# Autodesk Inventor assembly: Seed hand
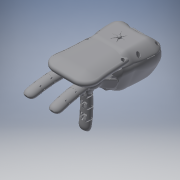
[picture p0: Inventor's stored thumbnail of the model, 180x180]
Saved by Autodesk Inventor 2016 (Build 200138000, 138)
## iProperties
Created: 2016-03-09
Part Number: Seed hand
Document SubType Name: Assembly
Designer: Ironic
Author: Ironic
## Documents named in this file (5)
- Z:\NICO\NICO_CAD_master\hand\Seed hand\Seed hand.iam
- Z:\NICO\NICO_CAD_master\hand\Seed hand\hand.ipt
- Z:\NICO\NICO_CAD_master\hand\Seed hand\forearm.ipt
- Z:\NICO\NICO_CAD_master\hand\Seed hand\finger_segment.ipt
- Z:\NICO\NICO_CAD_master\hand\Seed hand\fingertip.ipt
## Components (11 placed, 4 different names)
1. forearm:1 — Flush:1, Flush:2, Insert:4, Rotational:1
2. hand:1 — Insert:4, Insert:7, Insert:9, Rotational:1, Rotational:2, Rotational:5, Rotational:8
3. finger_segment:1 — Rotational:2, Rotational:3
4. finger_segment:2 — Insert:11, Rotational:3, Rotational:4
5. finger_segment:3 — Insert:7, Insert:8, Rotational:5, Rotational:6
6. finger_segment:4 — Insert:8, Insert:13, Rotational:6, Rotational:7
7. finger_segment:5 — Insert:9, Insert:10, Rotational:8, Rotational:9
8. finger_segment:6 — Insert:10, Insert:12, Rotational:9, Rotational:10
9. fingertip:1 — Insert:11, Rotational:4
10. fingertip:2 — Insert:13, Rotational:7
11. fingertip:3 — Insert:12, Rotational:10
## Relationships (20: RevoluteJoint 10, Insert 8, Flush 2)
- Flush:1: forearm:1
- Flush:2: forearm:1
- Insert:4: forearm:1 ↔ hand:1
- Insert:7 (-0.5 mm): hand:1 ↔ finger_segment:3
- Insert:8 (-0.5 mm): finger_segment:3 ↔ finger_segment:4
- Insert:9 (-0.5 mm): hand:1 ↔ finger_segment:5
- Insert:10 (-0.5 mm): finger_segment:5 ↔ finger_segment:6
- Insert:11 (0.5 mm): finger_segment:2 ↔ fingertip:1
- Insert:12 (0.5 mm): finger_segment:6 ↔ fingertip:3
- Insert:13 (0.5 mm): finger_segment:4 ↔ fingertip:2
- Rotational:1 [RevoluteJoint]: forearm:1 ↔ hand:1
- Rotational:2 [RevoluteJoint] (0.5 mm): hand:1 ↔ finger_segment:1
- Rotational:3 [RevoluteJoint] (0.5 mm): finger_segment:1 ↔ finger_segment:2
- Rotational:4 [RevoluteJoint] (0.5 mm): finger_segment:2 ↔ fingertip:1
- Rotational:5 [RevoluteJoint] (0.5 mm): hand:1 ↔ finger_segment:3
- Rotational:6 [RevoluteJoint] (0.5 mm): finger_segment:3 ↔ finger_segment:4
- Rotational:7 [RevoluteJoint] (0.5 mm): finger_segment:4 ↔ fingertip:2
- Rotational:8 [RevoluteJoint] (0.5 mm): hand:1 ↔ finger_segment:5
- Rotational:9 [RevoluteJoint] (0.5 mm): finger_segment:5 ↔ finger_segment:6
- Rotational:10 [RevoluteJoint] (0.5 mm): finger_segment:6 ↔ fingertip:3
